# Autodesk Inventor assembly: Lifting Chasis
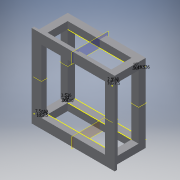
[picture p0: Inventor's stored thumbnail of the model, 180x180]
Saved by Autodesk Inventor 2016 (Build 200138000, 138)
## iProperties
Created: 2016-05-06
Part Number: Lifting Chasis
Document SubType Name: Assembly
Designer: Kenneth Daniel
Author: Kenneth Daniel
## Documents named in this file (6)
- C:\Users\Kenneth Daniel\Documents\Enes 100A\Final Prints and Versions\Lifting Chasis.iam
- C:\Users\Kenneth Daniel\Documents\Enes 100A\Lifting Chassis Work\Front Facing Beam Support.ipt
- C:\Users\Kenneth Daniel\Documents\Enes 100A\Lifting Chassis Work\Lower Beam Support.ipt
- C:\Users\Kenneth Daniel\Documents\Enes 100A\Lifting Chassis Work\Upper Beam Support.ipt
- C:\Users\Kenneth Daniel\Documents\Enes 100A\Lifting Chassis Work\Lower Beam Support_MIR1.ipt
- C:\Users\Kenneth Daniel\Documents\Enes 100A\Lifting Chassis Work\Upper Beam Support_MIR1.ipt
## Components (6 placed, 5 different names)
1. Front Facing Beam Support:1 — Flush:1, Flush:2, Mate:1, Flush:3, Flush:4, Mate:2
2. Front Facing Beam Support:2 — Mate:3, Flush:5, Flush:6
3. Lower Beam Support:1 — Flush:3, Flush:4, Mate:2, Flush:5
4. Upper Beam Support:1 — Flush:1, Flush:2, Mate:1, Mate:3, Flush:6
5. Lower Beam Support_MIR1:1
6. Upper Beam Support_MIR1:1
## Relationships (9: Flush 6, Mate 3)
- Flush:1: Front Facing Beam Support:1 ↔ Upper Beam Support:1
- Flush:2: Front Facing Beam Support:1 ↔ Upper Beam Support:1
- Mate:1: Front Facing Beam Support:1 ↔ Upper Beam Support:1
- Flush:3: Front Facing Beam Support:1 ↔ Lower Beam Support:1
- Flush:4: Front Facing Beam Support:1 ↔ Lower Beam Support:1
- Mate:2: Front Facing Beam Support:1 ↔ Lower Beam Support:1
- Mate:3: Front Facing Beam Support:2 ↔ Upper Beam Support:1
- Flush:5: Front Facing Beam Support:2 ↔ Lower Beam Support:1
- Flush:6: Front Facing Beam Support:2 ↔ Upper Beam Support:1
